# Autodesk Inventor assembly: Battery Conector
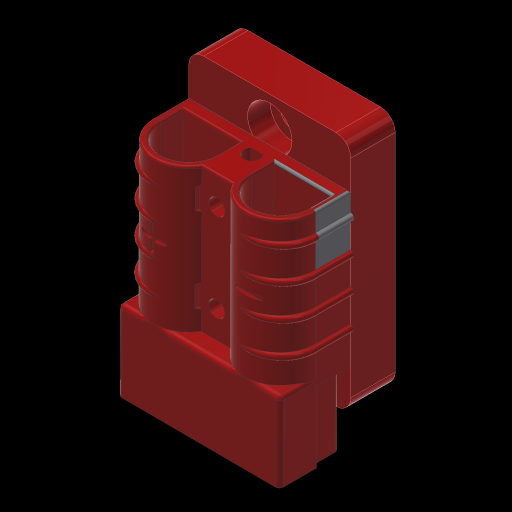
[picture p0: Inventor's stored thumbnail of the model, 512x512]
Saved by Autodesk Inventor 2023.3 (Build 273359000, 359)
## iProperties
Created: 2024-03-19
Part Number: Battery Conector
Document SubType Name: Assembly
Designer: mavericks
Author: mavericks
## Documents named in this file (3)
- C:\Users\mavericks\Desktop\Crescendo_2024-CAD\2024 Robot\COMMON PARTS\ELECTRONICS\Battery Conector.iam
- C:\Users\mavericks\Desktop\Crescendo_2024-CAD\2024 Robot\COMMON PARTS\ELECTRONICS\anderson battery connectorAnderson adapter.ipt
- C:\Users\mavericks\Desktop\Crescendo_2024-CAD\2024 Robot\COMMON PARTS\ELECTRONICS\anderson battery connectorAnderson_SB50_Connector_Updated.ipt
## Components (2 placed, 2 different names)
1. anderson battery connectorAnderson adapter:1 — Mate:1, Insert:1, Mate:2
2. anderson battery connectorAnderson_SB50_Connector_Updated:1 — Mate:1, Insert:1, Mate:2
## Relationships (3: Mate 2, Insert 1)
- Mate:1: anderson battery connectorAnderson adapter:1 ↔ anderson battery connectorAnderson_SB50_Connector_Updated:1
- Insert:1: anderson battery connectorAnderson adapter:1 ↔ anderson battery connectorAnderson_SB50_Connector_Updated:1
- Mate:2 (0.0762 mm): anderson battery connectorAnderson adapter:1 ↔ anderson battery connectorAnderson_SB50_Connector_Updated:1
